# Autodesk Inventor assembly: dial-indicator-holder-for-printing
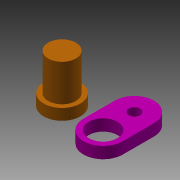
[picture p0: Inventor's stored thumbnail of the model, 180x180]
Saved by Autodesk Inventor 2014 (Build 180170000, 170)
## iProperties
Created: 2013-12-31
Part Number: dial-indicator-holder-for-printing
Document SubType Name: Assembly
Designer: caleb
Author: caleb
## Documents named in this file (3)
- C:\cygwin\home\caleb\caleb-typea-settings\designs\dial-gauge-holder\dial-indicator-holder-for-printing.iam
- C:\cygwin\home\caleb\caleb-typea-settings\designs\dial-gauge-holder\dial-indicator-holder-a.ipt
- C:\cygwin\home\caleb\caleb-typea-settings\designs\dial-gauge-holder\dial-indicator-holder-b.ipt
## Components (2 placed, 2 different names)
1. dial-indicator-holder-a:1 — Flush:2, Mate:4
2. dial-indicator-holder-b:1 — Flush:2
## Relationships (2: Flush 1, Mate 1)
- Flush:2: dial-indicator-holder-a:1 ↔ dial-indicator-holder-b:1
- Mate:4: dial-indicator-holder-a:1
